# Autodesk Inventor assembly: Front Upper Arm with pillow ball
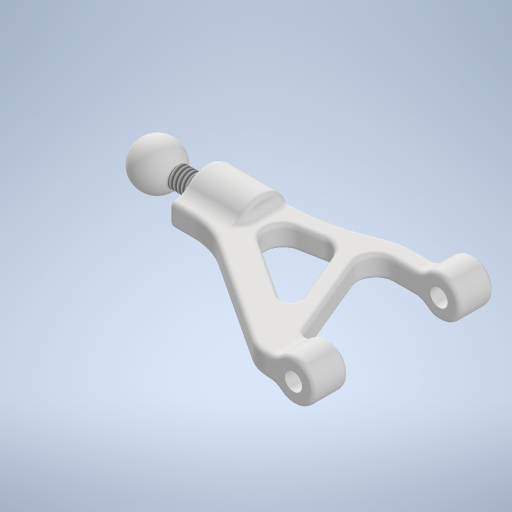
[picture p0: Inventor's stored thumbnail of the model, 512x512]
Saved by Autodesk Inventor 2024 (Build 280153000, 153)
## iProperties
Created: 2023-07-07
Part Number: Front Upper Arm with pillow ball
Document SubType Name: Assembly
Designer: birud
Author: birud
## Documents named in this file (3)
- C:\Users\birud\OneDrive\Desktop\Projects\EG\Front Upper Arm with pillow ball.iam
- C:\Users\birud\OneDrive\Desktop\Projects\EG\Front Upper ARM BP.ipt
- C:\Users\birud\OneDrive\Desktop\Projects\EG\Pillow Ball.ipt
## Components (2 placed, 2 different names)
1. Front Upper ARM BP:1 — Mate:1, Mate:2
2. Pillow Ball:1 — Mate:1, Mate:2
## Relationships (2: Mate 2)
- Mate:1: Front Upper ARM BP:1 ↔ Pillow Ball:1
- Mate:2 (88.9 mm): Front Upper ARM BP:1 ↔ Pillow Ball:1
